# Autodesk Inventor assembly: 4 Omni, Square_MIR1
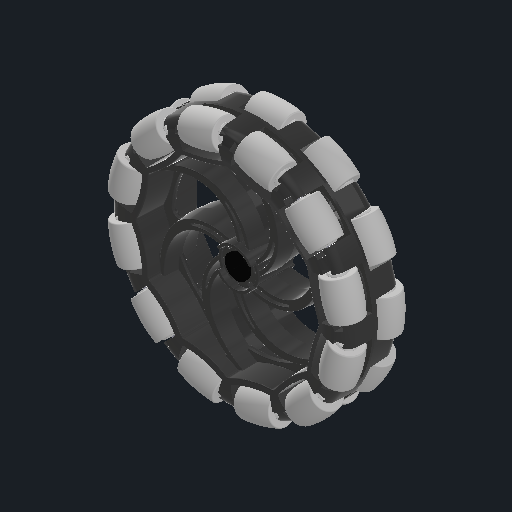
[picture p0: Inventor's stored thumbnail of the model, 512x512]
Saved by Autodesk Inventor 2023 (Build 270158000, 158)
## iProperties
Created: 2022-08-02
Part Number: 4 Omni, Square_MIR1
Document SubType Name: Assembly
Designer: Windows Macbook
Author: ylu12
## Documents named in this file (3)
- C:\Users\Windows Macbook\Desktop\VRC-SPIN-UP\Inventor\Motion\Wheels\Omni Wheel\4 Omni, Square_MIR1.iam
- C:\Users\Windows Macbook\Desktop\VRC-SPIN-UP\Inventor\Motion\Wheels\Reference Files\4 Omni_MIR1.ipt
- C:\Users\Windows Macbook\Desktop\VRC-SPIN-UP\Inventor\Motion\Insert Square_MIR1.ipt
## Components (3 placed, 2 different names)
1. 4 Omni_MIR1:1 — Flush:8, Mate:16, Mate:15
2. Insert Square_MIR1:1 — Flush:11, Flush:10, Mate:17
3. Insert Square_MIR1:2 — Angle:1, Mate:18, Flush:11, Flush:10, Flush:9
## Relationships (9: Flush 4, Mate 4, Angle 1)
- Flush:8: 4 Omni_MIR1:1
- Mate:16: 4 Omni_MIR1:1
- Mate:15: 4 Omni_MIR1:1
- Angle:1 (0 deg): Insert Square_MIR1:2
- Mate:18: Insert Square_MIR1:2
- Flush:11: Insert Square_MIR1:1 ↔ Insert Square_MIR1:2
- Flush:10: Insert Square_MIR1:1 ↔ Insert Square_MIR1:2
- Flush:9 [Mate] (7 mm): Insert Square_MIR1:2
- Mate:17 [Flush] (7.0104 mm): Insert Square_MIR1:1
